# Autodesk Inventor assembly: 몸
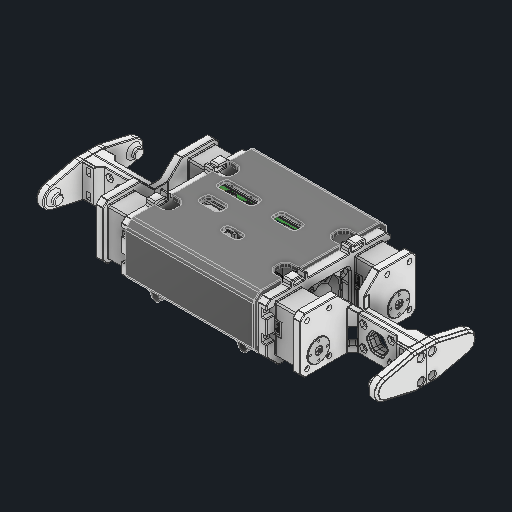
[picture p0: Inventor's stored thumbnail of the model, 512x512]
Saved by Autodesk Inventor 2027.1 (Build 311270010, 270A)
## iProperties
Created: 2026-08-12
Part Number: 몸
Document SubType Name: Assembly
Designer: moieboy9999
Mass: 499.031 g
Surface Area: 2413.88 cm^2
Volume: 364.423 cm^3
Density: 1.36937 g/cm^3
Author: moieboy9999
## Documents named in this file (4)
- D:\micro_dog_cad\몸\몸.iam
- D:\micro_dog_cad\몸\시스템\시스템조립.iam
- D:\micro_dog_cad\몸\프레임\프레임조립.iam
- D:\micro_dog_cad\몸\커버\몸커버.ipt
## Components (3 placed, 3 different names)
1. 시스템조립:1 [sub-assembly]
2. 프레임조립:1 [sub-assembly] — 메이트:3, 메이트:4, 메이트:5, 메이트:6, 메이트:7, 메이트:8
3. 몸커버:1 — 메이트:3, 메이트:4, 메이트:5
## Relationships (8: Mate 8)
- [Mate]: 시스템조립:1 ↔ 프레임조립:1
- [Mate]: 시스템조립:1 ↔ 프레임조립:1
- 메이트:3 [Mate]: 프레임조립:1 ↔ 몸커버:1
- 메이트:4 [Mate]: 프레임조립:1 ↔ 몸커버:1
- 메이트:5 [Mate]: 프레임조립:1 ↔ 몸커버:1
- 메이트:6 [Mate]: 프레임조립:1
- 메이트:7 [Mate]: 프레임조립:1
- 메이트:8 [Mate]: 프레임조립:1
